# Autodesk Inventor assembly: 000ASS_Bo_banh_xe_04
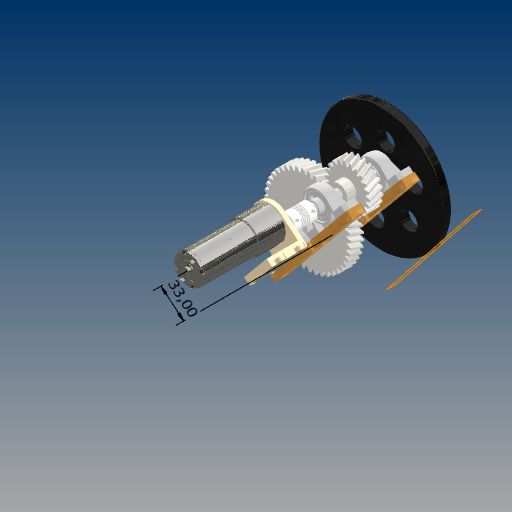
[picture p0: Inventor's stored thumbnail of the model, 512x512]
Saved by Autodesk Inventor 2021 (Build 250183000, 183)
## iProperties
Created: 2024-03-11
Part Number: 000ASS_Bo_banh_xe_04
Document SubType Name: Assembly
Designer: Admin
Author: Admin
## Documents named in this file (11)
- C:\Users\Admin\Desktop\DO_AN_TOT_NGHIEP_2024\Mechanical\Design_in_3D\Version_1\000ASS_Bo_banh_xe_04.iam
- C:\Users\Admin\Desktop\DO_AN_TOT_NGHIEP_2024\Mechanical\Design_in_3D\Library\kh-p-n-i-m-m-2.snapshot.1\khop-noi-mem.ipt
- C:\Users\Admin\Desktop\DO_AN_TOT_NGHIEP_2024\Mechanical\Design_in_3D\Version_1\02_Truc_02.ipt
- C:\Users\Admin\Desktop\DO_AN_TOT_NGHIEP_2024\Mechanical\Design_in_3D\Version_1\05_Banh_xe.ipt
- C:\Users\Admin\Desktop\DO_AN_TOT_NGHIEP_2024\Mechanical\Design_in_3D\Version_1\01_Truc_02.ipt
- C:\Users\Admin\Desktop\DO_AN_TOT_NGHIEP_2024\Mechanical\Design_in_3D\Library\kp000-1.snapshot.4\KP000\PK000.ipt
- C:\Users\Admin\Desktop\DO_AN_TOT_NGHIEP_2024\Mechanical\Design_in_3D\Library\Banh_rang\Banh_rang_bi_dan_03.ipt
- C:\Users\Admin\Desktop\DO_AN_TOT_NGHIEP_2024\Mechanical\Design_in_3D\Library\Banh_rang\Banh_rang_dan_03.ipt
- C:\Users\Admin\Desktop\DO_AN_TOT_NGHIEP_2024\Mechanical\Design_in_3D\Version_1\07_Mieng_go_bu_67x16.ipt
- C:\Users\Admin\Desktop\DO_AN_TOT_NGHIEP_2024\Mechanical\Design_in_3D\Library\DC_Servo_JGB37-520.iam
- C:\Users\Admin\Desktop\DO_AN_TOT_NGHIEP_2024\Mechanical\Design_in_3D\Library\08_Ga_dong_co.ipt
## Components (16 placed, 10 different names)
1. khop-noi-mem:1 — Mate:29, Mate:45
2. 02_Truc_02:1 — Mate:25, Flush:13, Mate:30, Mate:33, Mate:34, Mate:35, Flush:20
3. 05_Banh_xe:1 — Mate:25, Flush:13
4. 01_Truc_02:1 — Mate:29, Mate:30, Mate:31, Mate:32, Mate:36, Flush:21
5. PK000:1 — Mate:32, Flush:14, Flush:16, Flush:18, Mate:37, Flush:21, Insert:3, Mate:43
6. PK000:2 — Mate:31, Flush:14, Flush:17, Mate:38, Insert:2, Mate:44
7. PK000:3 — Mate:33, Flush:15, Flush:16, Flush:18, Insert:1, Mate:42
8. PK000:4 — Mate:34, Flush:15, Flush:17, Flush:20, Mate:39, Mate:40, Mate:41
9. Spur Gear2:1 — Mate:35, Flush:19
10. Spur Gear1:1 — Mate:36, Flush:19, Mate:37, Mate:38
11. 07_Mieng_go_bu_67x16:1 — Mate:39, Mate:40, Mate:41
12. 07_Mieng_go_bu_67x16:2 — Insert:3, Mate:43
13. 07_Mieng_go_bu_67x16:3 — Insert:2, Mate:44, Angle:1, Flush:22
14. 07_Mieng_go_bu_67x16:4 — Insert:1, Mate:42
15. DC_Servo_JGB37-520:1 [sub-assembly] — Mate:45, Angle:1, Mate:46, Mate:47, Mate:48
16. 08_Ga_dong_co:1 — Mate:46, Mate:47, Mate:48, Flush:22
## Relationships (35: Mate 21, Flush 10, Insert 3, Angle 1)
- Mate:25: 02_Truc_02:1 ↔ 05_Banh_xe:1
- Flush:13: 02_Truc_02:1 ↔ 05_Banh_xe:1
- Mate:29: khop-noi-mem:1 ↔ 01_Truc_02:1
- Mate:30 (70 mm): 02_Truc_02:1 ↔ 01_Truc_02:1
- Mate:31: 01_Truc_02:1 ↔ PK000:2
- Mate:32: 01_Truc_02:1 ↔ PK000:1
- Flush:14: PK000:1 ↔ PK000:2
- Mate:33: 02_Truc_02:1 ↔ PK000:3
- Mate:34: 02_Truc_02:1 ↔ PK000:4
- Flush:15: PK000:3 ↔ PK000:4
- Flush:16: PK000:1 ↔ PK000:3
- Flush:17: PK000:2 ↔ PK000:4
- Flush:18: PK000:1 ↔ PK000:3
- Mate:35: 02_Truc_02:1 ↔ Spur Gear2:1
- Mate:36: 01_Truc_02:1 ↔ Spur Gear1:1
- Flush:19: Spur Gear2:1 ↔ Spur Gear1:1
- Mate:37 (10 mm): PK000:1 ↔ Spur Gear1:1
- Mate:38 (10 mm): PK000:2 ↔ Spur Gear1:1
- Flush:20: 02_Truc_02:1 ↔ PK000:4
- Flush:21: 01_Truc_02:1 ↔ PK000:1
- Mate:39: PK000:4 ↔ 07_Mieng_go_bu_67x16:1
- Mate:40: PK000:4 ↔ 07_Mieng_go_bu_67x16:1
- Mate:41: PK000:4 ↔ 07_Mieng_go_bu_67x16:1
- Insert:1: PK000:3 ↔ 07_Mieng_go_bu_67x16:4
- Mate:42: PK000:3 ↔ 07_Mieng_go_bu_67x16:4
- Insert:2: PK000:2 ↔ 07_Mieng_go_bu_67x16:3
- Insert:3: PK000:1 ↔ 07_Mieng_go_bu_67x16:2
- Mate:43: PK000:1 ↔ 07_Mieng_go_bu_67x16:2
- Mate:44: PK000:2 ↔ 07_Mieng_go_bu_67x16:3
- Mate:45: khop-noi-mem:1 ↔ DC_Servo_JGB37-520:1
- Angle:1 (0 deg): 07_Mieng_go_bu_67x16:3 ↔ DC_Servo_JGB37-520:1
- Mate:46: DC_Servo_JGB37-520:1 ↔ 08_Ga_dong_co:1
- Mate:47: DC_Servo_JGB37-520:1 ↔ 08_Ga_dong_co:1
- Mate:48: DC_Servo_JGB37-520:1 ↔ 08_Ga_dong_co:1
- Flush:22: 07_Mieng_go_bu_67x16:3 ↔ 08_Ga_dong_co:1
